# Autodesk Inventor assembly: ALFA1
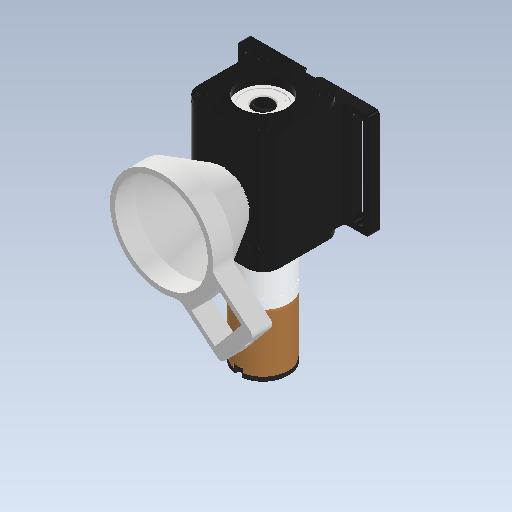
[picture p0: Inventor's stored thumbnail of the model, 512x512]
Saved by Autodesk Inventor 2020.2 (Build 242310000, 310)
## iProperties
Created: 2020-11-09
Part Number: ALFA1
Document SubType Name: Assembly
Designer: JK
Author: JK
## Documents named in this file (8)
- C:\Users\JK\Documents\Inventor\DispensadorPolvo\ALFA1.iam
- C:\Users\JK\Documents\Inventor\DispensadorPolvo\JGA25-372 24V Motor.ipt
- C:\Users\JK\Documents\Inventor\DispensadorPolvo\BRACKETXX.ipt
- C:\Users\JK\Documents\Inventor\DispensadorPolvo\Bearing.ipt
- C:\Users\JK\Documents\Inventor\DispensadorPolvo\TornilloDC.ipt
- C:\Users\JK\Documents\Inventor\DispensadorPolvo\CHute2.ipt
- C:\Users\JK\Documents\Inventor\DispensadorPolvo\soportemotor.ipt
- C:\Users\JK\Documents\Inventor\DispensadorPolvo\taparodamiento.ipt
## Components (7 placed, 7 different names)
1. JGA25-372 24V Motor:1 — Mate:17, Mate:18, Mate:19, Mate:22
2. BRACKETXX:1 — Mate:1, Mate:8, Mate:13, Mate:14, Mate:15, Mate:16, Mate:21, Mate:23, Mate:24
3. Bearing:1 — Mate:1, Mate:9, Mate:14
4. TornilloDC:1 — Mate:9
5. CHute2:1 — Mate:8
6. soportemotor:1 — Mate:15, Mate:16, Mate:17, Mate:18, Mate:19, Mate:24
7. taparodamiento:1 — Mate:21, Mate:22, Mate:23
## Relationships (14: Mate 14)
- Mate:1: BRACKETXX:1 ↔ Bearing:1
- Mate:8: BRACKETXX:1 ↔ CHute2:1
- Mate:9: Bearing:1 ↔ TornilloDC:1
- Mate:13: BRACKETXX:1
- Mate:14: BRACKETXX:1 ↔ Bearing:1
- Mate:15: BRACKETXX:1 ↔ soportemotor:1
- Mate:16: BRACKETXX:1 ↔ soportemotor:1
- Mate:17: JGA25-372 24V Motor:1 ↔ soportemotor:1
- Mate:18: JGA25-372 24V Motor:1 ↔ soportemotor:1
- Mate:19: JGA25-372 24V Motor:1 ↔ soportemotor:1
- Mate:21: BRACKETXX:1 ↔ taparodamiento:1
- Mate:22: JGA25-372 24V Motor:1 ↔ taparodamiento:1
- Mate:23: BRACKETXX:1 ↔ taparodamiento:1
- Mate:24: BRACKETXX:1 ↔ soportemotor:1
